# Autodesk Inventor assembly: Assemblyfull two pistons
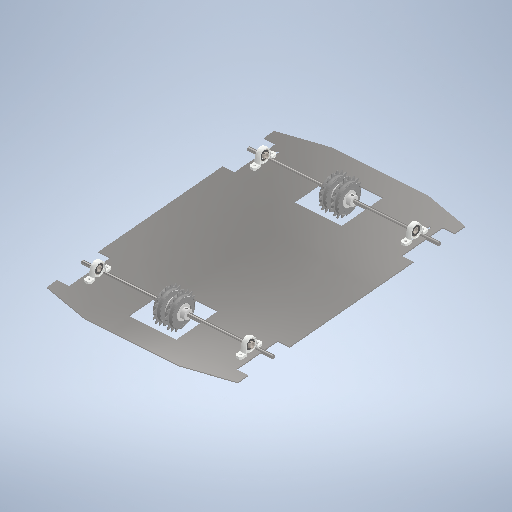
[picture p0: Inventor's stored thumbnail of the model, 512x512]
Saved by Autodesk Inventor 2026.1 (Build 301233020, 233B)
## iProperties
Created: 2026-01-22
Part Number: Assemblyfull two pistons
Document SubType Name: Assembly
Designer: user
Author: user
## Documents named in this file (4)
- D:\asu\machine element design\project\design\Assemblyfull two pistons .iam
- D:\asu\machine element design\project\design\chassis.ipt
- C:\Users\user\Downloads\pillow-block-bearing-p08-1.snapshot.17\Pillow Block P08\Pillow Block P08\Pillow Block P08.ipt
- D:\asu\machine element design\project\design\shaft assembly.iam
## Components (7 placed, 3 different names)
1. chassis:1 — Mate:1, Mate:2, Mate:3, Mate:4, Mate:5, Mate:6, Mate:7, Mate:8, Mate:9, Mate:10, Mate:11, Mate:12
2. Pillow Block P08:1 — Mate:1, Mate:2, Mate:3, Mate:14
3. Pillow Block P08:2 — Mate:5, Mate:11, Mate:12
4. Pillow Block P08:3 — Mate:6, Mate:7, Mate:8, Mate:13
5. Pillow Block P08:4 — Mate:4, Mate:9, Mate:10
6. shaft assembly:1 [sub-assembly] — Mate:13
7. shaft assembly:2 [sub-assembly] — Mate:14
## Relationships (14: Mate 14)
- Mate:1: chassis:1 ↔ Pillow Block P08:1
- Mate:2: chassis:1 ↔ Pillow Block P08:1
- Mate:3: chassis:1 ↔ Pillow Block P08:1
- Mate:4: chassis:1 ↔ Pillow Block P08:4
- Mate:5: chassis:1 ↔ Pillow Block P08:2
- Mate:6: chassis:1 ↔ Pillow Block P08:3
- Mate:7: chassis:1 ↔ Pillow Block P08:3
- Mate:8: chassis:1 ↔ Pillow Block P08:3
- Mate:9: chassis:1 ↔ Pillow Block P08:4
- Mate:10: chassis:1 ↔ Pillow Block P08:4
- Mate:11: chassis:1 ↔ Pillow Block P08:2
- Mate:12: chassis:1 ↔ Pillow Block P08:2
- Mate:13: Pillow Block P08:3 ↔ shaft assembly:1
- Mate:14: Pillow Block P08:1 ↔ shaft assembly:2
## Named parameters: sa_0 = 10000
note: some values were not read from the file. Shown as the stored number, unit unknown: "sa_0".
